# Autodesk Inventor assembly: bed
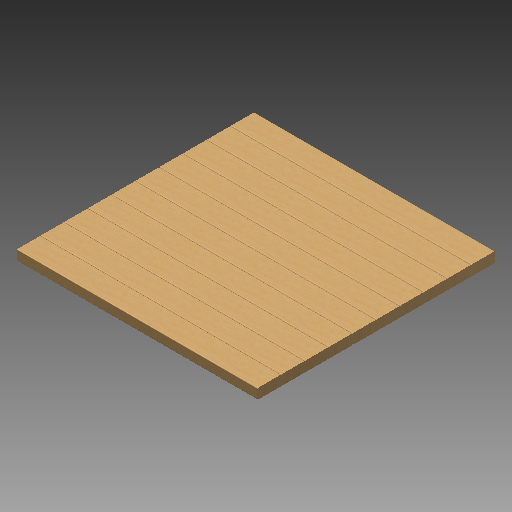
[picture p0: Inventor's stored thumbnail of the model, 512x512]
Saved by Autodesk Inventor 2019 (Build 230136000, 136)
## iProperties
Created: 2019-05-07
Part Number: bed
Document SubType Name: Assembly
Designer: Alex Jones
Author: Alex Jones
## Documents named in this file (2)
- C:\Users\Alex Jones\Documents\Inventor\CNC\bed.iam
- C:\Users\Alex Jones\Documents\Inventor\CNC\2x4.ipt
## Components (10 placed, 1 different names)
1. 2x4:1 — Flush:9, Flush:10, Flush:11, Flush:12, Mate:4, Mate:5
2. 2x4:2 — Flush:11, Flush:12, Flush:13, Flush:14, Mate:3, Mate:4
3. 2x4:3 — Flush:13, Flush:14, Flush:15, Flush:16, Mate:2, Mate:3
4. 2x4:4 — Flush:15, Flush:16, Flush:17, Flush:18, Mate:1, Mate:2
5. 2x4:5 — Flush:17, Flush:18, Mate:1
6. 2x4:6 — Flush:5, Flush:6, Flush:7, Flush:8, Mate:6, Mate:7
7. 2x4:7 — Flush:7, Flush:8, Flush:9, Flush:10, Mate:5, Mate:6
8. 2x4:8 — Flush:1, Flush:2, Flush:5, Flush:6, Mate:7, Mate:8
9. 2x4:9 — Flush:1, Flush:2, Flush:3, Flush:4, Mate:8, Mate:9
10. 2x4:10 — Flush:3, Flush:4, Mate:9
## Relationships (27: Flush 18, Mate 9)
- Flush:1: 2x4:8 ↔ 2x4:9
- Flush:2: 2x4:8 ↔ 2x4:9
- Flush:3: 2x4:9 ↔ 2x4:10
- Flush:4: 2x4:9 ↔ 2x4:10
- Flush:5: 2x4:6 ↔ 2x4:8
- Flush:6: 2x4:6 ↔ 2x4:8
- Flush:7: 2x4:6 ↔ 2x4:7
- Flush:8: 2x4:6 ↔ 2x4:7
- Flush:9: 2x4:1 ↔ 2x4:7
- Flush:10: 2x4:1 ↔ 2x4:7
- Flush:11: 2x4:1 ↔ 2x4:2
- Flush:12: 2x4:1 ↔ 2x4:2
- Flush:13: 2x4:2 ↔ 2x4:3
- Flush:14: 2x4:2 ↔ 2x4:3
- Flush:15: 2x4:3 ↔ 2x4:4
- Flush:16: 2x4:3 ↔ 2x4:4
- Flush:17: 2x4:4 ↔ 2x4:5
- Flush:18: 2x4:4 ↔ 2x4:5
- Mate:1: 2x4:4 ↔ 2x4:5
- Mate:2: 2x4:3 ↔ 2x4:4
- Mate:3: 2x4:2 ↔ 2x4:3
- Mate:4: 2x4:1 ↔ 2x4:2
- Mate:5: 2x4:1 ↔ 2x4:7
- Mate:6: 2x4:6 ↔ 2x4:7
- Mate:7: 2x4:6 ↔ 2x4:8
- Mate:8: 2x4:8 ↔ 2x4:9
- Mate:9: 2x4:9 ↔ 2x4:10
